# Autodesk Inventor assembly: board2.brd
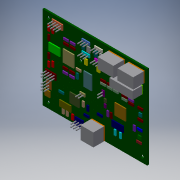
[picture p0: Inventor's stored thumbnail of the model, 180x180]
Saved by Autodesk Inventor 2016 (Build 200138000, 138)
## iProperties
Created: 2016-03-25
Part Number: board2.brd
Document SubType Name: Assembly
Designer: Paschalis
Sending System: Autodesk Inventor 2016
Preprocessor: ST-DEVELOPER v16.1
Title: C:\Users\Paschalis\Documents\eagle\Measuring-PCB\3D\board2.brd.stp
Author: Paschalis
## Documents named in this file (44)
- C:\Users\Paschalis\Documents\eagle\Measuring-PCB\3D\board2.brd.iam
- C:\Users\Paschalis\Documents\eagle\Measuring-PCB\3D\board2.brd_Outline.ipt
- C:\Users\Paschalis\Documents\eagle\Measuring-PCB\3D\PHOENIX-TERMINAL-3PIN, PHOENIX-TERMINAL-3PIN_1.ipt
- C:\Users\Paschalis\Documents\eagle\Measuring-PCB\3D\SOT95P280X145-6N, ADR3425ARJZ-R7_3.ipt
- C:\Users\Paschalis\Documents\eagle\Measuring-PCB\3D\SOP65P780X200-28N, ADS1256IDBT_5.ipt
- C:\Users\Paschalis\Documents\eagle\Measuring-PCB\3D\SOIC127P1032X265-16N, ADUM5000ARWZ_7.ipt
- C:\Users\Paschalis\Documents\eagle\Measuring-PCB\3D\1X02, AIN6-7_1X02_9.ipt
- C:\Users\Paschalis\Documents\eagle\Measuring-PCB\3D\TQFP32-08, ATMEGA328P_TQFP_11.ipt
- C:\Users\Paschalis\Documents\eagle\Measuring-PCB\3D\BATTCON_12MM, 3V_13.ipt
- C:\Users\Paschalis\Documents\eagle\Measuring-PCB\3D\C3216, 10U_15.ipt
- C:\Users\Paschalis\Documents\eagle\Measuring-PCB\3D\C3216, 0_1U_17.ipt
- C:\Users\Paschalis\Documents\eagle\Measuring-PCB\3D\C3216, 47U_19.ipt
- C:\Users\Paschalis\Documents\eagle\Measuring-PCB\3D\C3216, 100P_22.ipt
- C:\Users\Paschalis\Documents\eagle\Measuring-PCB\3D\C3216, 18P_26.ipt
- C:\Users\Paschalis\Documents\eagle\Measuring-PCB\3D\C3216, 1U_47.ipt
- C:\Users\Paschalis\Documents\eagle\Measuring-PCB\3D\C3216, 10N_49.ipt
- C:\Users\Paschalis\Documents\eagle\Measuring-PCB\3D\C3216, 2_2U_51.ipt
- C:\Users\Paschalis\Documents\eagle\Measuring-PCB\3D\C3216, 22P_53.ipt
- C:\Users\Paschalis\Documents\eagle\Measuring-PCB\3D\DS3234, DS3234_58.ipt
- C:\Users\Paschalis\Documents\eagle\Measuring-PCB\3D\PAS_5X20, 15A_60.ipt
- C:\Users\Paschalis\Documents\eagle\Measuring-PCB\3D\2X3, FEMALE_62.ipt
- C:\Users\Paschalis\Documents\eagle\Measuring-PCB\3D\2X04, ISOLATED_CON_2X04_64.ipt
- C:\Users\Paschalis\Documents\eagle\Measuring-PCB\3D\1X03, JP1A_1X03_66.ipt
- C:\Users\Paschalis\Documents\eagle\Measuring-PCB\3D\1X03, JP1B_1X03_68.ipt
- C:\Users\Paschalis\Documents\eagle\Measuring-PCB\3D\1X03, JP2A_1X03_70.ipt
- C:\Users\Paschalis\Documents\eagle\Measuring-PCB\3D\1X03, JP2B_1X03_72.ipt
- C:\Users\Paschalis\Documents\eagle\Measuring-PCB\3D\SOT95P280X145-5N, LP2985-33DBVT_74.ipt
- C:\Users\Paschalis\Documents\eagle\Measuring-PCB\3D\SOIC-16, IC_DIL16-SOIC-16_76.ipt
- C:\Users\Paschalis\Documents\eagle\Measuring-PCB\3D\2X04, NON-ISOLATED_CON_2X04_78.ipt
- C:\Users\Paschalis\Documents\eagle\Measuring-PCB\3D\HC49U-V, 7_68MHZ_80.ipt
- C:\Users\Paschalis\Documents\eagle\Measuring-PCB\3D\HC49U-V, 16MHZ_82.ipt
- C:\Users\Paschalis\Documents\eagle\Measuring-PCB\3D\LVK25, 0_005_84.ipt
- C:\Users\Paschalis\Documents\eagle\Measuring-PCB\3D\R3216, 4_7K_86.ipt
- C:\Users\Paschalis\Documents\eagle\Measuring-PCB\3D\M3216, 560K_88.ipt
- C:\Users\Paschalis\Documents\eagle\Measuring-PCB\3D\M3216, 5_49M_90.ipt
- C:\Users\Paschalis\Documents\eagle\Measuring-PCB\3D\M3216, 1K_95.ipt
- C:\Users\Paschalis\Documents\eagle\Measuring-PCB\3D\R3216, 100_100.ipt
- C:\Users\Paschalis\Documents\eagle\Measuring-PCB\3D\R3216, 10K_104.ipt
- C:\Users\Paschalis\Documents\eagle\Measuring-PCB\3D\TACTILE-SWITCH-SMD, TAC_SWITCHSMD_108.ipt
- C:\Users\Paschalis\Documents\eagle\Measuring-PCB\3D\1X02, RX-TX_1X02_110.ipt
- C:\Users\Paschalis\Documents\eagle\Measuring-PCB\3D\SJ, SJ1-RST_SJ_112.ipt
- C:\Users\Paschalis\Documents\eagle\Measuring-PCB\3D\SJ, SJ2-SYNC_SJ_114.ipt
- C:\Users\Paschalis\Documents\eagle\Measuring-PCB\3D\2TERMINALBLOCK_10MMPITCH, 2PIN_TERMINAL_PCBMOUNT_116.ipt
- C:\Users\Paschalis\Documents\eagle\Measuring-PCB\3D\connectors.ipt
## Components (79 placed, 79 different names)
1. board2.brd_Outline:1
2. 1WIRE-BUS_2
3. ADR3425_4
4. ADS1256_6
5. ADUM5000_8
6. AIN6-7_10
7. ATMEGA328_12
8. BAT1_14 — Flush:2
9. C1_16
10. C2_18
11. C3_20
12. C4_21
13. C5_23
14. C6_24
15. C7_25
16. C8_27
17. C9_28
18. C10_29
19. C11_30
20. C12_31
21. C13_32
22. C14_33
23. C15_34
24. C16_35
25. C17_36
26. C18_37
27. C19_38
28. C20_39
29. C21_40
30. C22_41
31. C23_42
32. C24_43
33. C25_44
34. C26_45
35. C27_46
36. C28_48
37. C29_50
38. C30_52
39. C31_54
40. C32_55
41. C33_56
42. C34_57
43. DS3234_59
44. F1_61 — Flush:4
45. 2X3_63
46. ISOLATED_CON_65 — Flush:3
47. JP1A_67
48. JP1B_69
49. JP2A_71
50. JP2B_73
51. LP2985_75
52. MAX14850_77
53. NON-ISOLATED_CON_79
54. Q1_81
55. Q2_83
56. R1_85
57. R2_87
58. R2A40_89
59. R2A400_91
60. R2B40_92
61. R2B400_93
62. R3_94
63. R3A_96
64. R3B_97
65. R4_98
66. R5_99
67. R6_101
68. R7_102
69. R8_103
70. R9_105
71. R10_106
72. R11_107
73. RESET_109
74. RX-TX_111
75. SJ1-RST_113
76. SJ2-SYNC_115
77. VOUT_117 — Flush:1
78. VPANEL_118
79. connectors:1 — Flush:1, Flush:2, Flush:3, Flush:4
## Relationships (4: Flush 4)
- Flush:1: VOUT_117 ↔ connectors:1
- Flush:2: BAT1_14 ↔ connectors:1
- Flush:3: ISOLATED_CON_65 ↔ connectors:1
- Flush:4: F1_61 ↔ connectors:1
